# Autodesk Inventor assembly: Target
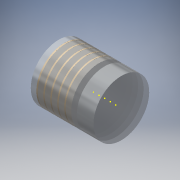
[picture p0: Inventor's stored thumbnail of the model, 180x180]
Saved by Autodesk Inventor 2017 (Build 210142000, 142)
## iProperties
Created: 2017-02-26
Part Number: Target
Document SubType Name: Assembly
Designer: Jake
Author: Jake
## Documents named in this file (3)
- C:\Users\Jake\Documents\5thYear\Project\CAD\Target.iam
- C:\Users\Jake\Documents\5thYear\Project\CAD\Compound Layer.iam
- C:\Users\Jake\Documents\5thYear\Project\CAD\Vinyltoluene.ipt
## Components (10 placed, 2 different names)
1. Compound Layer:1 [sub-assembly] — Mate:1, Mate:3, Mate:4, Mate:5
2. Compound Layer:2 [sub-assembly] — Mate:2, Mate:6, Mate:7, Mate:8
3. Compound Layer:3 [sub-assembly] — Mate:2, Mate:3, Mate:5, Mate:6
4. Compound Layer:4 [sub-assembly] — Mate:7, Mate:8, Mate:9, Mate:10
5. Compound Layer:5 [sub-assembly] — Mate:1, Mate:4
6. Vinyltoluene:1 — Mate:9, Mate:10, Mate:11, Mate:12
7. Vinyltoluene:2 — Mate:11, Mate:12, Mate:13, Mate:14
8. Vinyltoluene:3 — Mate:13, Mate:14, Mate:15, Mate:16
9. Vinyltoluene:4 — Mate:15, Mate:16, Mate:17, Mate:18
10. Vinyltoluene:5 — Mate:17, Mate:18
## Relationships (18: Mate 18)
- Mate:1: Compound Layer:1 ↔ Compound Layer:5
- Mate:2: Compound Layer:2 ↔ Compound Layer:3
- Mate:3: Compound Layer:1 ↔ Compound Layer:3
- Mate:4: Compound Layer:1 ↔ Compound Layer:5
- Mate:5: Compound Layer:1 ↔ Compound Layer:3
- Mate:6: Compound Layer:2 ↔ Compound Layer:3
- Mate:7: Compound Layer:2 ↔ Compound Layer:4
- Mate:8: Compound Layer:2 ↔ Compound Layer:4
- Mate:9: Compound Layer:4 ↔ Vinyltoluene:1
- Mate:10: Compound Layer:4 ↔ Vinyltoluene:1
- Mate:11: Vinyltoluene:1 ↔ Vinyltoluene:2
- Mate:12: Vinyltoluene:1 ↔ Vinyltoluene:2
- Mate:13: Vinyltoluene:2 ↔ Vinyltoluene:3
- Mate:14: Vinyltoluene:2 ↔ Vinyltoluene:3
- Mate:15: Vinyltoluene:3 ↔ Vinyltoluene:4
- Mate:16: Vinyltoluene:3 ↔ Vinyltoluene:4
- Mate:17: Vinyltoluene:4 ↔ Vinyltoluene:5
- Mate:18: Vinyltoluene:4 ↔ Vinyltoluene:5
